# Autodesk Inventor assembly: ROVassembly
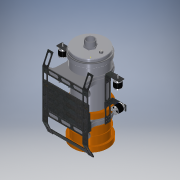
[picture p0: Inventor's stored thumbnail of the model, 180x180]
Saved by Autodesk Inventor 2016 (Build 200138000, 138)
## iProperties
Created: 2015-10-11
Part Number: ROVassembly
Document SubType Name: Assembly
Designer: Artur
Mass: 1358.92 g
Surface Area: 5794.57 cm^2
Volume: 799.87 cm^3
Density: 1.69892 g/cm^3
Author: Artur
## Documents named in this file (31)
- C:\Users\Artur\Dropbox\stuff\ROV_current\ROVassembly.iam
- C:\Users\Artur\Dropbox\stuff\ROV_current\hullPipe.ipt
- C:\Users\Artur\Dropbox\stuff\ROV_current\ArduinoUno.ipt
- C:\Users\Artur\Dropbox\stuff\ROV_current\ESC.ipt
- C:\Users\Artur\Dropbox\stuff\ROV_current\transverse.ipt
- C:\Users\Artur\Dropbox\stuff\ROV_current\arduinoShelf.ipt
- C:\Users\Artur\Dropbox\stuff\ROV_current\usbRangeExtender.ipt
- C:\Users\Artur\Dropbox\stuff\ROV_current\camera.ipt
- C:\Users\Artur\Dropbox\stuff\ROV_current\Motor.ipt
- C:\Users\Artur\Dropbox\stuff\ROV_current\usbHubSmall.ipt
- C:\Users\Artur\Dropbox\stuff\ROV_current\miniRelay.ipt
- C:\Users\Artur\Dropbox\stuff\ROV_current\aftPlug.ipt
- C:\Users\Artur\Dropbox\stuff\ROV_current\PVCConnectorFemale3_4inch.ipt
- C:\Users\Artur\Dropbox\stuff\ROV_current\frameMount.ipt
- C:\Users\Artur\Dropbox\stuff\ROV_current\plexiglassWindow.ipt
- C:\Users\Artur\Dropbox\stuff\ROV_current\transverseClipStiffener.ipt
- C:\Users\Artur\Dropbox\stuff\ROV_current\sled.ipt
- C:\Users\Artur\Dropbox\stuff\ROV_current\30PSIPressureSensor.ipt
- C:\Users\Artur\Dropbox\stuff\ROV_current\doubleSocketPipe.ipt
- C:\Users\Artur\Dropbox\stuff\ROV_current\PVCConnectorMale3_4inch.ipt
- C:\Users\Artur\Dropbox\stuff\ROV_current\socketBracket.ipt
- C:\Users\Artur\Dropbox\stuff\ROV_current\motorBracket.ipt
- C:\Users\Artur\Dropbox\stuff\ROV_current\brushlessMotorControlBoard.ipt
- C:\Users\Artur\Dropbox\stuff\ROV_current\sideLongitudinal.ipt
- C:\Users\Artur\Dropbox\stuff\ROV_current\ballastBar.ipt
- C:\Users\Artur\Dropbox\stuff\ROV_current\longitudinal - top.ipt
- C:\Users\Artur\Dropbox\stuff\ROV_current\longitudinal - bottom.ipt
- C:\Users\Artur\Dropbox\stuff\ROV_current\ROVassembly.ElectronicsHarness.iam
- C:\Users\Artur\Dropbox\stuff\ROV_current\CommonGNDVDD.ipt
- C:\Users\Artur\Dropbox\stuff\ROV_current\fwdPlug.ipt
- C:\Users\Artur\Dropbox\stuff\ROV_current\ballastBarSmall.ipt
## Components (71 placed, 30 different names)
1. hullPipe:1 — Flush:264, Tangent:3, Tangent:4, Mate:288, Mate:289
2. longitudinal - bottom:2 — Angle:1, Mate:7, Mate:13, Flush:14, Flush:19, Flush:20, Mate:17, Flush:23, Flush:24, Mate:20, Flush:28, Flush:29, Flush:30, Flush:32, Flush:33, Flush:34, Flush:35, Flush:39, Mate:32, Flush:42, Flush:72, Angle:2, Mate:97, Flush:87, Flush:88, Flush:89, Flush:90, Mate:99, Mate:100, Mate:140, Mate:141, Mate:142, Flush:94, Flush:262, Mate:284
3. longitudinal - bottom:1 — Flush:31, Flush:32, Flush:33, Mate:26, Flush:37, Mate:89, Mate:90, Mate:93, Mate:94, Flush:93, Tangent:4
4. longitudinal - top:1 — Flush:37, Mate:29, Flush:39, Mate:34, Flush:43, Mate:95, Mate:150, Tangent:3
5. longitudinal - top:2 — Flush:34, Flush:35, Flush:38, Mate:27, Flush:40, Mate:30, Flush:41, Mate:91, Mate:92, Mate:96, Mate:101, Flush:91, Flush:92, Angle:12, Angle:15, Flush:103, Mate:200, Flush:104, Flush:263, Flush:264
6. transverse:1 — Flush:28, Mate:32, Mate:33, Flush:42
7. transverse:2 — Flush:24, Mate:30, Flush:41, Mate:31, Mate:35, Mate:60
8. transverse:3 — Mate:20, Flush:40, Mate:31, Mate:33
9. transverse:4 — Mate:34, Mate:35, Flush:43, Mate:63
10. transverse:5 — Flush:30, Mate:26, Mate:28
11. transverse:6 — Flush:20, Mate:17, Mate:18, Mate:24, Flush:38
12. transverse:7 — Mate:24, Flush:29, Mate:27, Mate:28, Mate:29
13. transverse:8 — Mate:7, Flush:19, Flush:23, Mate:18, Flush:31, Angle:9, Angle:10, Angle:13
14. arduinoShelf:1 — Mate:13, Flush:14, Mate:15, Flush:15, Flush:16, Mate:16, Mate:36, Mate:50, Mate:51, Flush:73, Flush:74, Mate:64, Mate:65, Flush:75, Mate:186, Flush:94, Flush:96, Flush:98, Flush:100, Flush:102, Mate:258, Mate:259, Flush:106, Flush:107
15. ArduinoUno:1 — Mate:15, Flush:15, Flush:16
16. ESC:1 — Mate:16, Flush:95, Flush:97
17. ESC:2 — Mate:36, Flush:95, Flush:96, Flush:97, Flush:98
18. ESC:3 — Mate:50, Flush:99, Flush:101, Flush:102
19. ESC:4 — Mate:51, Flush:99, Flush:100, Flush:101
20. usbRangeExtender:1 — Flush:73, Flush:74, Mate:64, Mate:66
21. camera:1 — Flush:72, Mate:60, Mate:63
22. Motor:1 — Mate:175, Mate:176, Angle:19
23. Motor:2 — Mate:173, Mate:174, Angle:18
24. Motor:3 — Mate:177, Mate:178, Angle:17
25. Motor:4 — Mate:171, Mate:172, Angle:20
26. usbHubSmall:1 — Mate:65, Mate:66, Flush:75
27. miniRelay:1 — Mate:201, Mate:216, Angle:29
28. miniRelay:2 — Mate:202, Mate:211, Angle:28
29. miniRelay:3 — Mate:208, Mate:209, Angle:31
30. miniRelay:4 — Mate:207, Mate:210, Angle:30
31. miniRelay:5 — Mate:206, Mate:213, Angle:27
32. miniRelay:6 — Mate:205, Mate:212, Angle:26
33. miniRelay:7 — Mate:204, Mate:214, Angle:25
34. miniRelay:8 — Mate:203, Mate:215
35. aftPlug:1 — Mate:220, Mate:221, Mate:222, Mate:223, Mate:224, Angle:32, Mate:284, Mate:289
36. PVCConnectorFemale3_4inch:1 — Angle:2, Angle:9, Mate:154, Mate:223
37. frameMount:1 — Mate:97, Flush:90, Mate:99, Mate:102
38. frameMount:2 — Flush:87, Mate:102, Mate:150
39. frameMount:3 — Mate:96, Flush:89, Mate:100
40. frameMount:4 — Mate:95, Flush:88, Mate:101
41. frameMount:5 — Mate:91, Mate:92, Flush:91
42. frameMount:6 — Mate:93, Mate:94, Flush:93
43. frameMount:7 — Mate:89, Mate:90, Flush:92
44. plexiglassWindow:1 — Mate:285, Mate:286, Mate:287
45. transverseClipStiffener:1 — Mate:134, Mate:135, Mate:159, Mate:160, Mate:161, Angle:34, Angle:35
46. transverseClipStiffener:2 — Mate:195, Mate:196, Mate:197, Mate:278, Mate:279
47. sled:1 — Mate:134, Mate:166, Angle:35, Mate:279
48. sled:2 — Mate:135, Mate:167, Angle:34, Mate:273, Mate:278, Mate:294, Flush:265, Flush:266, Flush:267, Flush:268, Flush:269, Flush:270, Mate:300, Mate:301, Mate:306, Flush:271, Flush:272
49. 30PSIPressureSensor:1 — Angle:13, Mate:220, Mate:221
50. doubleSocketPipe:1 — Flush:263, Mate:288, Mate:290, Mate:291, Mate:292, Mate:293
51. PVCConnectorMale3_4inch:1 — Mate:154, Angle:10, Mate:222, Mate:224
52. socketBracket:2 — Angle:12, Mate:159, Mate:160, Mate:161, Mate:166, Mate:167, Mate:282, Mate:283, Tangent:1, Tangent:2
53. socketBracket:3 — Angle:15, Mate:195, Mate:196, Mate:197, Mate:273, Mate:280, Mate:281, Mate:292, Mate:293, Mate:298, Mate:307, Mate:308
54. motorBracket:1 — Mate:177, Mate:178, Angle:17, Mate:245, Mate:271, Mate:272
55. motorBracket:2 — Mate:175, Mate:176, Angle:19, Mate:242, Mate:269, Mate:270
56. motorBracket:3 — Mate:173, Mate:174, Angle:18, Mate:239, Mate:276, Mate:277
57. motorBracket:4 — Mate:171, Mate:172, Angle:20, Mate:236, Mate:274, Mate:275
58. brushlessMotorControlBoard:1 — Flush:103, Mate:200, Mate:201, Mate:202, Mate:203, Mate:204, Mate:205, Mate:206, Mate:207, Mate:208, Mate:209, Mate:210, Mate:211, Mate:212, Mate:213, Mate:214, Mate:215, Mate:216, Angle:25, Angle:26, Angle:27, Angle:28, Angle:29, Angle:30, Angle:31, Mate:217, Flush:104
59. sideLongitudinal:1 — Mate:236, Mate:242, Mate:269, Mate:270, Mate:274, Mate:275, Mate:280, Mate:283, Tangent:1
60. sideLongitudinal:2 — Mate:239, Mate:245, Mate:271, Mate:272, Mate:276, Mate:277, Mate:281, Mate:282, Tangent:2
61. ROVassembly.ElectronicsHarness [sub-assembly]
62. CommonGNDVDD:1 — Mate:259, Flush:106, Mate:260, Flush:262
63. CommonGNDVDD:2 — Mate:258, Flush:107, Mate:260
64. fwdPlug:1 — Mate:285, Mate:286, Mate:287, Mate:290, Mate:291
65. ballastBarSmall:1 — Mate:306, Flush:271, Flush:272
66. ballastBar:1 — Mate:294, Mate:295, Flush:265, Mate:307, Mate:309
67. ballastBar:2 — Mate:295, Mate:296, Flush:266, Mate:308, Mate:310
68. ballastBar:3 — Mate:296, Flush:267, Mate:298
69. ballastBar:4 — Flush:268, Mate:300, Mate:302, Mate:309, Mate:311
70. ballastBar:5 — Flush:269, Mate:301, Mate:311
71. ballastBar:6 — Flush:270, Mate:302, Mate:310
## Relationships (213: Mate 131, Flush 57, Angle 21, Tangent 4)
- Angle:1 (0 deg): longitudinal - bottom:2
- Mate:7: longitudinal - bottom:2 ↔ transverse:8
- Mate:13: longitudinal - bottom:2 ↔ arduinoShelf:1
- Flush:14: longitudinal - bottom:2 ↔ arduinoShelf:1
- Mate:15 (5 mm): arduinoShelf:1 ↔ ArduinoUno:1
- Flush:15 (15 mm): arduinoShelf:1 ↔ ArduinoUno:1
- Flush:16: arduinoShelf:1 ↔ ArduinoUno:1
- Mate:16: arduinoShelf:1 ↔ ESC:1
- Flush:19: longitudinal - bottom:2 ↔ transverse:8
- Flush:20: longitudinal - bottom:2 ↔ transverse:6
- Mate:17: longitudinal - bottom:2 ↔ transverse:6
- Flush:23 (25 mm): longitudinal - bottom:2 ↔ transverse:8
- Mate:18: transverse:6 ↔ transverse:8
- Flush:24: longitudinal - bottom:2 ↔ transverse:2
- Mate:20: longitudinal - bottom:2 ↔ transverse:3
- Flush:28: longitudinal - bottom:2 ↔ transverse:1
- Mate:24: transverse:6 ↔ transverse:7
- Flush:29: longitudinal - bottom:2 ↔ transverse:7
- Flush:30: longitudinal - bottom:2 ↔ transverse:5
- Flush:31: longitudinal - bottom:1 ↔ transverse:8
- Flush:32: longitudinal - bottom:2 ↔ longitudinal - bottom:1
- Flush:33: longitudinal - bottom:2 ↔ longitudinal - bottom:1
- Flush:34: longitudinal - bottom:2 ↔ longitudinal - top:2
- Flush:35: longitudinal - bottom:2 ↔ longitudinal - top:2
- Mate:26: longitudinal - bottom:1 ↔ transverse:5
- Flush:37: longitudinal - bottom:1 ↔ longitudinal - top:1
- Flush:38: longitudinal - top:2 ↔ transverse:6
- Mate:27: longitudinal - top:2 ↔ transverse:7
- Mate:28: transverse:5 ↔ transverse:7
- Mate:29: longitudinal - top:1 ↔ transverse:7
- Flush:39: longitudinal - bottom:2 ↔ longitudinal - top:1
- Flush:40: longitudinal - top:2 ↔ transverse:3
- Mate:30: longitudinal - top:2 ↔ transverse:2
- Flush:41: longitudinal - top:2 ↔ transverse:2
- Mate:31: transverse:2 ↔ transverse:3
- Mate:32: longitudinal - bottom:2 ↔ transverse:1
- Mate:33: transverse:1 ↔ transverse:3
- Flush:42: longitudinal - bottom:2 ↔ transverse:1
- Mate:34: longitudinal - top:1 ↔ transverse:4
- Mate:35: transverse:2 ↔ transverse:4
- Flush:43: longitudinal - top:1 ↔ transverse:4
- Mate:36: arduinoShelf:1 ↔ ESC:2
- Mate:50: arduinoShelf:1 ↔ ESC:3
- Mate:51: arduinoShelf:1 ↔ ESC:4
- Flush:72 (10 mm): longitudinal - bottom:2 ↔ camera:1
- Mate:60: transverse:2 ↔ camera:1
- Flush:73 (-20 mm): arduinoShelf:1 ↔ usbRangeExtender:1
- Flush:74 (25 mm): arduinoShelf:1 ↔ usbRangeExtender:1
- Mate:63: transverse:4 ↔ camera:1
- Mate:64: arduinoShelf:1 ↔ usbRangeExtender:1
- Mate:65: arduinoShelf:1 ↔ usbHubSmall:1
- Mate:66 (20 mm): usbRangeExtender:1 ↔ usbHubSmall:1
- Flush:75 (-8 mm): arduinoShelf:1 ↔ usbHubSmall:1
- Angle:2 (0 deg): longitudinal - bottom:2 ↔ PVCConnectorFemale3_4inch:1
- Mate:89: longitudinal - bottom:1 ↔ frameMount:7
- Mate:90: longitudinal - bottom:1 ↔ frameMount:7
- Mate:91: longitudinal - top:2 ↔ frameMount:5
- Mate:92: longitudinal - top:2 ↔ frameMount:5
- Mate:93: longitudinal - bottom:1 ↔ frameMount:6
- Mate:94: longitudinal - bottom:1 ↔ frameMount:6
- Mate:95: longitudinal - top:1 ↔ frameMount:4
- Mate:96: longitudinal - top:2 ↔ frameMount:3
- Mate:97: longitudinal - bottom:2 ↔ frameMount:1
- Flush:87: longitudinal - bottom:2 ↔ frameMount:2
- Flush:88: longitudinal - bottom:2 ↔ frameMount:4
- Flush:89: longitudinal - bottom:2 ↔ frameMount:3
- Flush:90: longitudinal - bottom:2 ↔ frameMount:1
- Mate:99: longitudinal - bottom:2 ↔ frameMount:1
- Mate:100: longitudinal - bottom:2 ↔ frameMount:3
- Mate:101: longitudinal - top:2 ↔ frameMount:4
- Mate:102: frameMount:1 ↔ frameMount:2
- Mate:134: transverseClipStiffener:1 ↔ sled:1
- Mate:135: transverseClipStiffener:1 ↔ sled:2
- Mate:140: longitudinal - bottom:2
- Mate:141: longitudinal - bottom:2
- Mate:142: longitudinal - bottom:2
- Flush:91: longitudinal - top:2 ↔ frameMount:5
- Flush:92: longitudinal - top:2 ↔ frameMount:7
- Flush:93: longitudinal - bottom:1 ↔ frameMount:6
- Mate:150: longitudinal - top:1 ↔ frameMount:2
- Angle:9 (0 deg): transverse:8 ↔ PVCConnectorFemale3_4inch:1
- Mate:154: PVCConnectorFemale3_4inch:1 ↔ PVCConnectorMale3_4inch:1
- Angle:10 (0 deg): transverse:8 ↔ PVCConnectorMale3_4inch:1
- Angle:12 (180 deg): longitudinal - top:2 ↔ socketBracket:2
- Mate:159: transverseClipStiffener:1 ↔ socketBracket:2
- Mate:160: transverseClipStiffener:1 ↔ socketBracket:2
- Mate:161: transverseClipStiffener:1 ↔ socketBracket:2
- Mate:166: sled:1 ↔ socketBracket:2
- Mate:167: sled:2 ↔ socketBracket:2
- Angle:13 (0 deg): transverse:8 ↔ 30PSIPressureSensor:1
- Mate:171: Motor:4 ↔ motorBracket:4
- Mate:172: Motor:4 ↔ motorBracket:4
- Mate:173: Motor:2 ↔ motorBracket:3
- Mate:174: Motor:2 ↔ motorBracket:3
- Mate:175: Motor:1 ↔ motorBracket:2
- Mate:176: Motor:1 ↔ motorBracket:2
- Mate:177: Motor:3 ↔ motorBracket:1
- Mate:178: Motor:3 ↔ motorBracket:1
- Mate:186: arduinoShelf:1
- Flush:94 (135 mm): longitudinal - bottom:2 ↔ arduinoShelf:1
- Flush:95 (-9 mm): ESC:1 ↔ ESC:2
- Flush:96 (10 mm): arduinoShelf:1 ↔ ESC:2
- Flush:97: ESC:1 ↔ ESC:2
- Flush:98 (80 mm): arduinoShelf:1 ↔ ESC:2
- Flush:99 (9 mm): ESC:3 ↔ ESC:4
- Flush:100 (10 mm): arduinoShelf:1 ↔ ESC:4
- Flush:101: ESC:3 ↔ ESC:4
- Flush:102 (98 mm): arduinoShelf:1 ↔ ESC:3
- Angle:15 (180 deg): longitudinal - top:2 ↔ socketBracket:3
- Angle:17 (180 deg): Motor:3 ↔ motorBracket:1
- Angle:18 (180 deg): Motor:2 ↔ motorBracket:3
- Angle:19 (180 deg): Motor:1 ↔ motorBracket:2
- Angle:20 (180 deg): Motor:4 ↔ motorBracket:4
- Mate:195: transverseClipStiffener:2 ↔ socketBracket:3
- Mate:196: transverseClipStiffener:2 ↔ socketBracket:3
- Mate:197: transverseClipStiffener:2 ↔ socketBracket:3
- Flush:103: longitudinal - top:2 ↔ brushlessMotorControlBoard:1
- Mate:200: longitudinal - top:2 ↔ brushlessMotorControlBoard:1
- Mate:201: miniRelay:1 ↔ brushlessMotorControlBoard:1
- Mate:202: miniRelay:2 ↔ brushlessMotorControlBoard:1
- Mate:203: miniRelay:8 ↔ brushlessMotorControlBoard:1
- Mate:204: miniRelay:7 ↔ brushlessMotorControlBoard:1
- Mate:205: miniRelay:6 ↔ brushlessMotorControlBoard:1
- Mate:206: miniRelay:5 ↔ brushlessMotorControlBoard:1
- Mate:207: miniRelay:4 ↔ brushlessMotorControlBoard:1
- Mate:208: miniRelay:3 ↔ brushlessMotorControlBoard:1
- Mate:209: miniRelay:3 ↔ brushlessMotorControlBoard:1
- Mate:210: miniRelay:4 ↔ brushlessMotorControlBoard:1
- Mate:211: miniRelay:2 ↔ brushlessMotorControlBoard:1
- Mate:212: miniRelay:6 ↔ brushlessMotorControlBoard:1
- Mate:213: miniRelay:5 ↔ brushlessMotorControlBoard:1
- Mate:214: miniRelay:7 ↔ brushlessMotorControlBoard:1
- Mate:215: miniRelay:8 ↔ brushlessMotorControlBoard:1
- Mate:216: miniRelay:1 ↔ brushlessMotorControlBoard:1
- Angle:25 (0 deg): miniRelay:7 ↔ brushlessMotorControlBoard:1
- Angle:26 (0 deg): miniRelay:6 ↔ brushlessMotorControlBoard:1
- Angle:27 (0 deg): miniRelay:5 ↔ brushlessMotorControlBoard:1
- Angle:28 (0 deg): miniRelay:2 ↔ brushlessMotorControlBoard:1
- Angle:29 (0 deg): miniRelay:1 ↔ brushlessMotorControlBoard:1
- Angle:30 (0 deg): miniRelay:4 ↔ brushlessMotorControlBoard:1
- Angle:31 (0 deg): miniRelay:3 ↔ brushlessMotorControlBoard:1
- Mate:217: brushlessMotorControlBoard:1
- Mate:220: aftPlug:1 ↔ 30PSIPressureSensor:1
- Mate:221: aftPlug:1 ↔ 30PSIPressureSensor:1
- Mate:222: aftPlug:1 ↔ PVCConnectorMale3_4inch:1
- Mate:223: aftPlug:1 ↔ PVCConnectorFemale3_4inch:1
- Mate:224: aftPlug:1 ↔ PVCConnectorMale3_4inch:1
- Angle:32 (0 deg): aftPlug:1
- Mate:236: motorBracket:4 ↔ sideLongitudinal:1
- Mate:239: motorBracket:3 ↔ sideLongitudinal:2
- Mate:242: motorBracket:2 ↔ sideLongitudinal:1
- Mate:245: motorBracket:1 ↔ sideLongitudinal:2
- Flush:104 (-130 mm): longitudinal - top:2 ↔ brushlessMotorControlBoard:1
- Angle:34 (0 deg): transverseClipStiffener:1 ↔ sled:2
- Angle:35 (0 deg): transverseClipStiffener:1 ↔ sled:1
- Mate:258: arduinoShelf:1 ↔ CommonGNDVDD:2
- Mate:259: arduinoShelf:1 ↔ CommonGNDVDD:1
- Flush:106 (-6 mm): arduinoShelf:1 ↔ CommonGNDVDD:1
- Flush:107 (6 mm): arduinoShelf:1 ↔ CommonGNDVDD:2
- Mate:260: CommonGNDVDD:1 ↔ CommonGNDVDD:2
- Flush:262 (220 mm): longitudinal - bottom:2 ↔ CommonGNDVDD:1
- Mate:269: motorBracket:2 ↔ sideLongitudinal:1
- Mate:270: motorBracket:2 ↔ sideLongitudinal:1
- Mate:271: motorBracket:1 ↔ sideLongitudinal:2
- Mate:272: motorBracket:1 ↔ sideLongitudinal:2
- Mate:273: sled:2 ↔ socketBracket:3
- Mate:274: motorBracket:4 ↔ sideLongitudinal:1
- Mate:275: motorBracket:4 ↔ sideLongitudinal:1
- Mate:276: motorBracket:3 ↔ sideLongitudinal:2
- Mate:277: motorBracket:3 ↔ sideLongitudinal:2
- Mate:278: transverseClipStiffener:2 ↔ sled:2
- Mate:279: transverseClipStiffener:2 ↔ sled:1
- Mate:280: socketBracket:3 ↔ sideLongitudinal:1
- Mate:281: socketBracket:3 ↔ sideLongitudinal:2
- Mate:282: socketBracket:2 ↔ sideLongitudinal:2
- Mate:283: socketBracket:2 ↔ sideLongitudinal:1
- Tangent:1: socketBracket:2 ↔ sideLongitudinal:1
- Tangent:2: socketBracket:2 ↔ sideLongitudinal:2
- Mate:284: longitudinal - bottom:2 ↔ aftPlug:1
- Mate:285: plexiglassWindow:1 ↔ fwdPlug:1
- Mate:286 (-15 mm): plexiglassWindow:1 ↔ fwdPlug:1
- Mate:287 (-15 mm): plexiglassWindow:1 ↔ fwdPlug:1
- Flush:263: longitudinal - top:2 ↔ doubleSocketPipe:1
- Flush:264: hullPipe:1 ↔ longitudinal - top:2
- Tangent:3: hullPipe:1 ↔ longitudinal - top:1
- Tangent:4: hullPipe:1 ↔ longitudinal - bottom:1
- Mate:288: hullPipe:1 ↔ doubleSocketPipe:1
- Mate:289: hullPipe:1 ↔ aftPlug:1
- Mate:290: doubleSocketPipe:1 ↔ fwdPlug:1
- Mate:291: doubleSocketPipe:1 ↔ fwdPlug:1
- Mate:292: doubleSocketPipe:1 ↔ socketBracket:3
- Mate:293: doubleSocketPipe:1 ↔ socketBracket:3
- Mate:294: sled:2 ↔ ballastBar:1
- Mate:295: ballastBar:1 ↔ ballastBar:2
- Mate:296: ballastBar:2 ↔ ballastBar:3
- Mate:298: socketBracket:3 ↔ ballastBar:3
- Flush:265: sled:2 ↔ ballastBar:1
- Flush:266: sled:2 ↔ ballastBar:2
- Flush:267: sled:2 ↔ ballastBar:3
- Flush:268: sled:2 ↔ ballastBar:4
- Flush:269: sled:2 ↔ ballastBar:5
- Flush:270: sled:2 ↔ ballastBar:6
- Mate:300: sled:2 ↔ ballastBar:4
- Mate:301: sled:2 ↔ ballastBar:5
- Mate:302: ballastBar:4 ↔ ballastBar:6
- Mate:306: sled:2 ↔ ballastBarSmall:1
- Flush:271: sled:2 ↔ ballastBarSmall:1
- Flush:272: sled:2 ↔ ballastBarSmall:1
- Mate:307: socketBracket:3 ↔ ballastBar:1
- Mate:308: socketBracket:3 ↔ ballastBar:2
- Mate:309: ballastBar:1 ↔ ballastBar:4
- Mate:310: ballastBar:2 ↔ ballastBar:6
- Mate:311: ballastBar:4 ↔ ballastBar:5
